# Autodesk Inventor assembly: Gear2_LargeAndSmall
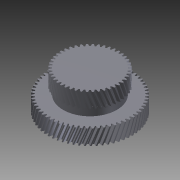
[picture p0: Inventor's stored thumbnail of the model, 180x180]
Saved by Autodesk Inventor 2012 (Build 160160000, 160)
## iProperties
Created: 2011-10-22
Part Number: Gear2_LargeAndSmall
Document SubType Name: Assembly
Designer: KuttaA
Author: KuttaA
## Documents named in this file (3)
- C:\Users\KuttaA\Dropbox\Hexapod Research\Leg Design\Other Parts\Intermediary Gear Box\Gear2_LargeAndSmall.iam
- C:\Users\KuttaA\Dropbox\Hexapod Research\Leg Design\Other Parts\Intermediary Gear Box\LargeGear.ipt
- C:\Users\KuttaA\Dropbox\Hexapod Research\Leg Design\Other Parts\Intermediary Gear Box\SmallGear.ipt
## Components (2 placed, 2 different names)
1. Spur Gear2:1 — Mate:2, Mate:3, Mate:4
2. Spur Gear1:1 — Mate:2, Mate:3, Mate:4
## Relationships (3: Mate 3)
- Mate:2: Spur Gear2:1 ↔ Spur Gear1:1
- Mate:3: Spur Gear2:1 ↔ Spur Gear1:1
- Mate:4: Spur Gear2:1 ↔ Spur Gear1:1
